# Autodesk Inventor assembly: ShootingMech_BeltAssembly
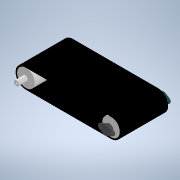
[picture p0: Inventor's stored thumbnail of the model, 180x180]
Saved by Autodesk Inventor 2020 (Build 240168000, 168)
## iProperties
Created: 2022-01-27
Part Number: ShootingMech_BeltAssembly
Document SubType Name: Assembly
Designer: danie
Author: danie
## Documents named in this file (6)
- C:\Users\danie\Documents\Capstone\Solidworks\ShootingMech_BeltAssembly.iam
- C:\Users\danie\Documents\Capstone\Solidworks\Shooting_Belt_2.ipt
- C:\Users\danie\Documents\Capstone\Solidworks\ShootingMech_Roller.ipt
- C:\Users\danie\Documents\Capstone\Solidworks\1327K108_Rotary Shaft.ipt
- C:\Users\danie\Documents\Capstone\Solidworks\4575N32_Light Duty Mounted Ball Bearing.ipt
- C:\Users\danie\Documents\Capstone\Solidworks\ShootingMech_MotorCoupling2.ipt
## Components (9 placed, 5 different names)
1. Shooting_Belt_2:1 — Rigid:1, Rotational:1, Cylindrical:1, Cylindrical:2
2. ShootingMech_Roller:1 — Rigid:1, Rotational:5
3. ShootingMech_Roller:2 — Rotational:1
4. 1327K108_Rotary Shaft:1 — Cylindrical:1, Rotational:4
5. 1327K108_Rotary Shaft:2 — Cylindrical:2, Rotational:2, Rotational:3
6. 4575N32_Light Duty Mounted Ball Bearing:1 — Rotational:3
7. 4575N32_Light Duty Mounted Ball Bearing:2 — Rotational:2
8. 4575N32_Light Duty Mounted Ball Bearing:3 — Rotational:4
9. ShootingMech_MotorCoupling2:1 — Rotational:5
## Relationships (8: RevoluteJoint 5, CylindricalJoint 2, WeldJoint 1)
- Rigid:1 [WeldJoint]: Shooting_Belt_2:1 ↔ ShootingMech_Roller:1
- Rotational:1 [RevoluteJoint]: Shooting_Belt_2:1 ↔ ShootingMech_Roller:2
- Cylindrical:1: Shooting_Belt_2:1 ↔ 1327K108_Rotary Shaft:1
- Cylindrical:2: Shooting_Belt_2:1 ↔ 1327K108_Rotary Shaft:2
- Rotational:2 [RevoluteJoint]: 1327K108_Rotary Shaft:2 ↔ 4575N32_Light Duty Mounted Ball Bearing:2
- Rotational:3 [RevoluteJoint]: 1327K108_Rotary Shaft:2 ↔ 4575N32_Light Duty Mounted Ball Bearing:1
- Rotational:4 [RevoluteJoint]: 1327K108_Rotary Shaft:1 ↔ 4575N32_Light Duty Mounted Ball Bearing:3
- Rotational:5 [RevoluteJoint] (-1.27 mm): ShootingMech_Roller:1 ↔ ShootingMech_MotorCoupling2:1
